# Autodesk Inventor assembly: CassingHardware
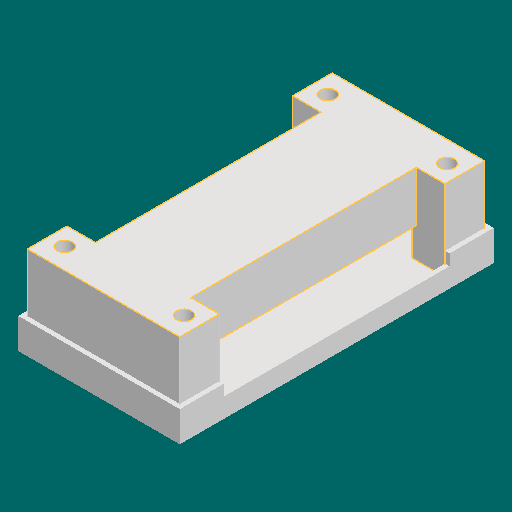
[picture p0: Inventor's stored thumbnail of the model, 512x512]
Saved by Autodesk Inventor 2025.2 (Build 292293000, 293)
## iProperties
Created: 2025-04-22
Part Number: CassingHardware
Document SubType Name: Assembly
Designer: ia088
Author: ia088
## Documents named in this file (3)
- C:\Users\ia088\OneDrive\Dokumen\2matkul_sem4\mikrokontroler\mikro\Tugas_Mikro\Mekanik\CassingHardware.iam
- C:\Users\ia088\OneDrive\Dokumen\2matkul_sem4\mikrokontroler\mikro\Tugas_Mikro\Mekanik\atas.ipt
- C:\Users\ia088\OneDrive\Dokumen\2matkul_sem4\mikrokontroler\mikro\Tugas_Mikro\Mekanik\bawah.ipt
## Components (2 placed, 2 different names)
1. atas:1 — Flush:1, Flush:2
2. bawah:1 — Flush:1, Flush:2
## Relationships (2: Flush 2)
- Flush:1: atas:1 ↔ bawah:1
- Flush:2: atas:1 ↔ bawah:1
